# Autodesk Inventor assembly: Calosc(podstawa do poprawy)
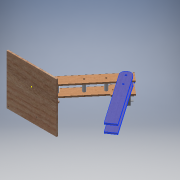
[picture p0: Inventor's stored thumbnail of the model, 180x180]
Saved by Autodesk Inventor 2017 (Build 210142000, 142)
## iProperties
Part Number: Calosc(podstawa do poprawy)
Material: Ogólny
Document SubType Name: Assembly
Designer: Damian
Author: Damian
## Documents named in this file (4)
- C:\Users\Damian\Documents\Inventor\Nowe\2.0\Calosc(podstawa do poprawy).iam
- C:\Users\Damian\Documents\Inventor\Nowe\2.0\podstawa.ipt
- C:\Users\Damian\Documents\Inventor\Nowe\2.0\Segment_1.iam
- C:\Users\Damian\Documents\Inventor\Nowe\2.0\Segment_2.iam
## Components (3 placed, 3 different names)
1. podstawa:1 — Wstaw:1
2. Segment_1:1 [sub-assembly] — Wstaw:1, Wstaw:2
3. Segment_2:1 [sub-assembly] — Wstaw:2
## Relationships (2: Insert 2)
- Wstaw:1 [Insert]: podstawa:1 ↔ Segment_1:1
- Wstaw:2 [Insert]: Segment_1:1 ↔ Segment_2:1
